# Autodesk Inventor assembly: Armbracket-Base
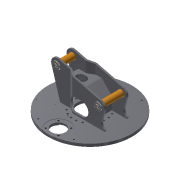
[picture p0: Inventor's stored thumbnail of the model, 180x180]
Saved by Autodesk Inventor 2022 Beta2 (Build 260130000, 130) ContinuousBuild 0
## iProperties
Shininess: 0.0
Length Units: 11269
Angle Units: 11279
Time Units: 11290
Mass Units: 11283
Length Display Precision: 3
Angle Display Precision: 2
Part Number: Armbracket-Base
Document SubType Name: Assembly
Description: Armbracket
Designer: Joe M
Engineer: Joe M
Created: 2016-01-21
Density: 0.0
Volume: 0.0
Area: 0.0
PropertySet Name: Model Information
Control State: 0
Master: False
Checked Out: False
Title: Arminfästning
Author: Joe M
## Documents named in this file (7)
- C:\Autodesk Inventor 2021 Intro Practice Files\BOM\Armbracket-Base.iam
- C:\Autodesk Inventor 2021 Intro Practice Files\BOM\3136 1149 25.iam
- C:\Autodesk Inventor 2021 Intro Practice Files\BOM\3136 7044 74.ipt
- C:\Autodesk Inventor 2021 Intro Practice Files\BOM\3136 7044 91.ipt
- C:\Autodesk Inventor 2021 Intro Practice Files\BOM\3136 7044 79.ipt
- C:\Autodesk Inventor 2021 Intro Practice Files\BOM\3136 7057 14.ipt
- C:\Autodesk Inventor 2021 Intro Practice Files\BOM\0301 2344 00.ipt
## Components (12 placed, 6 different names)
1. 0301 2344 00:19 — Insert:15
2. 3136 1149 25:1 [sub-assembly] — Insert:5, Insert:6, Insert:15
3. 3136 7044 74:1 — Insert:5, Insert:9, Insert:10
4. 3136 7044 91:1 — Insert:6, Insert:7, Insert:8
5. 3136 7044 79:1 — Insert:7, Insert:36
6. 3136 7044 79:2 — Insert:8, Insert:33
7. 3136 7044 79:3 — Insert:9, Insert:34
8. 3136 7044 79:4 — Insert:10, Insert:35
9. 3136 7057 14:1 — Insert:33
10. 3136 7057 14:2 — Insert:34
11. 3136 7057 14:3 — Insert:35
12. 3136 7057 14:4 — Insert:36
## Relationships (11: Insert 11)
- Insert:5 (-2 mm): 3136 1149 25:1 ↔ 3136 7044 74:1
- Insert:6: 3136 1149 25:1 ↔ 3136 7044 91:1
- Insert:7 (0.5 mm): 3136 7044 91:1 ↔ 3136 7044 79:1
- Insert:8 (0.5 mm): 3136 7044 91:1 ↔ 3136 7044 79:2
- Insert:9 (0.5 mm): 3136 7044 74:1 ↔ 3136 7044 79:3
- Insert:10 (0.5 mm): 3136 7044 74:1 ↔ 3136 7044 79:4
- Insert:15: 0301 2344 00:19 ↔ 3136 1149 25:1
- Insert:33: 3136 7044 79:2 ↔ 3136 7057 14:1
- Insert:34: 3136 7044 79:3 ↔ 3136 7057 14:2
- Insert:35: 3136 7044 79:4 ↔ 3136 7057 14:3
- Insert:36: 3136 7044 79:1 ↔ 3136 7057 14:4
